# Autodesk Inventor assembly: 8T_CAM
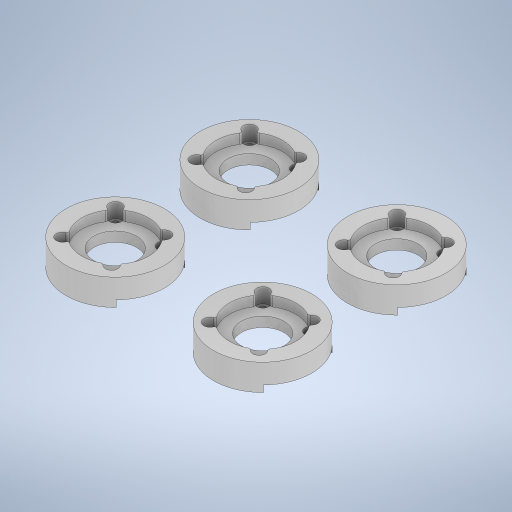
[picture p0: Inventor's stored thumbnail of the model, 512x512]
Saved by Autodesk Inventor 2024.2 (Build 282272000, 272)
## iProperties
Created: 2024-01-12
Part Number: 8T_CAM
Document SubType Name: Assembly
Designer: chanh
Author: chanh
## Documents named in this file (3)
- C:\Users\chanh\내 드라이브\로봇\Humanoid\Roboin Humanoid Project\Inventor\rh_plus_7_axis_robot_arm_hardware\CAM\8T\8T_CAM.iam
- C:\Users\chanh\내 드라이브\로봇\Humanoid\Roboin Humanoid Project\Inventor\rh_plus_7_axis_robot_arm_hardware\CAM\8T\axis_4_top_frame.ipt
- C:\Users\chanh\내 드라이브\로봇\Humanoid\Roboin Humanoid Project\Inventor\rh_plus_7_axis_robot_arm_hardware\CAM\8T\axis_6_top_frame.ipt
## Components (4 placed, 2 different names)
1. axis_4_top_frame:1 — Mate:1, Mate:2, Flush:1, Mate:3, Flush:2, Flush:3, Flush:6, Flush:7, Flush:8
2. axis_6_top_frame:1 — Mate:3, Flush:2, Flush:3
3. axis_4_top_frame:2 — Flush:6, Flush:7, Flush:8
4. axis_6_top_frame:2
## Relationships (12: Flush 8, Mate 4)
- Mate:1: axis_4_top_frame:1
- Mate:2: axis_4_top_frame:1
- Flush:1: axis_4_top_frame:1
- Mate:3 (-20 mm): axis_4_top_frame:1 ↔ axis_6_top_frame:1
- Flush:2: axis_4_top_frame:1 ↔ axis_6_top_frame:1
- Flush:3: axis_4_top_frame:1 ↔ axis_6_top_frame:1
- [Mate] (-20 mm): axis_4_top_frame:2 ↔ axis_6_top_frame:2
- [Flush]: axis_4_top_frame:2 ↔ axis_6_top_frame:2
- [Flush]: axis_4_top_frame:2 ↔ axis_6_top_frame:2
- Flush:6 (45 mm): axis_4_top_frame:1 ↔ axis_4_top_frame:2
- Flush:7: axis_4_top_frame:1 ↔ axis_4_top_frame:2
- Flush:8: axis_4_top_frame:1 ↔ axis_4_top_frame:2
## Named parameters: d6_d3 = -20 mm, d7_d4 = 0 mm, d8_d5 = 0 mm
